# Autodesk Inventor assembly: pc053_33
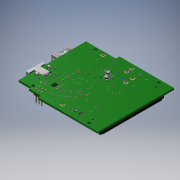
[picture p0: Inventor's stored thumbnail of the model, 180x180]
Saved by Autodesk Inventor 2017 (Build 210142000, 142)
## iProperties
Created: 2016-10-24
Part Number: pc053_33
Document SubType Name: Assembly
Designer: phpgb
Author: phpgb
## Documents named in this file (3)
- P:\cad\designs\uob-hep-pc053a\trunk\design_files\worklib\pc053a_toplevel\physical\3DModel\pc053_33.iam
- P:\cad\designs\uob-hep-pc053a\trunk\design_files\worklib\pc053a_toplevel\physical\3DModel\pc053a_toplevel_33.iam
- P:\cad\steps_files\FMCblankFrontPanel10.ipt
## Components (2 placed, 2 different names)
1. pc053a_toplevel_33:1 [sub-assembly] — Mate:1, Mate:2, Angle:1
2. FMCblankFrontPanel10:1 — Mate:1, Mate:2, Angle:1
## Relationships (3: Mate 2, Angle 1)
- Mate:1: pc053a_toplevel_33:1 ↔ FMCblankFrontPanel10:1
- Mate:2: pc053a_toplevel_33:1 ↔ FMCblankFrontPanel10:1
- Angle:1 (0 deg): pc053a_toplevel_33:1 ↔ FMCblankFrontPanel10:1
